# Autodesk Inventor assembly: ASY Рама №3 платформа
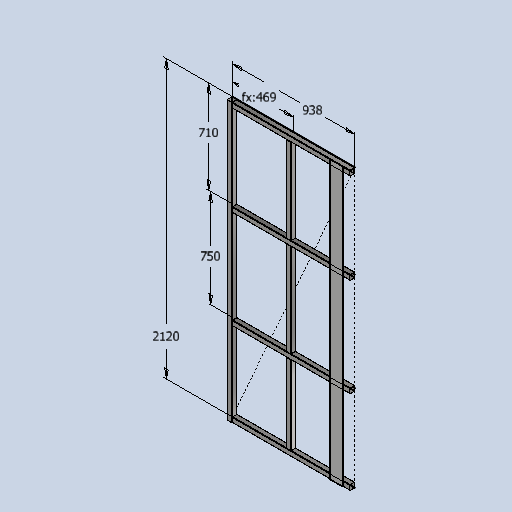
[picture p0: Inventor's stored thumbnail of the model, 512x512]
Saved by Autodesk Inventor 2025.1 (Build 291241020, 241B)
## iProperties
_SolveAssemblyDoc: Frame Generator Solve Assembly
_Version: 25.0.0
Created: 2025-01-19
Part Number: ASY Рама №3 платформа
Document SubType Name: Assembly
Designer: pokla
Author: pokla
## Documents named in this file (4)
- C:\Users\user\YandexDisk-badmisterfox\home pc\Inventor\NDM-VOS_powder_hopper\ASY Рама №3 платформа.iam
- C:\Users\user\YandexDisk-badmisterfox\home pc\Inventor\NDM-VOS_powder_hopper\ASY Рама №3 платформа.ipt
- C:\Users\user\YandexDisk-badmisterfox\home pc\Inventor\NDM-VOS_powder_hopper\ASY Рама №3 платформа1.ipt
- C:\Users\user\YandexDisk-badmisterfox\home pc\Inventor\NDM-VOS_powder_hopper\ASY Рама №3 платформа\Frame\Frame 1737401537000.iam
## Components (3 placed, 2 different names)
1. ASY Рама №3 платформа:1
2. ASY Рама №3 платформа:2 — Mate:1, Flush:1, Flush:2
3. Frame 1737401537000:1 [sub-assembly] — Mate:1, Flush:1, Flush:2
## Relationships (3: Flush 2, Mate 1)
- Mate:1: ASY Рама №3 платформа:2 ↔ Frame 1737401537000:1
- Flush:1: ASY Рама №3 платформа:2 ↔ Frame 1737401537000:1
- Flush:2 (50 mm): ASY Рама №3 платформа:2 ↔ Frame 1737401537000:1
